# Autodesk Inventor assembly: WheelAssembly3.0
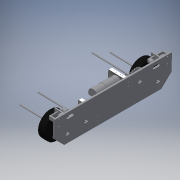
[picture p0: Inventor's stored thumbnail of the model, 180x180]
Saved by Autodesk Inventor 2017 (Build 210142000, 142)
## iProperties
Created: 2017-07-22
Part Number: WheelAssembly3.0
Document SubType Name: Assembly
Designer: User
Author: User
## Documents named in this file (13)
- C:\Robotics\CAD\WheelAssembly3.0.iam
- C:\Robotics\CAD\2016-17_CAD\DriveTrain\DriveTrain3.0.ipt
- C:\Robotics\CAD\COTSParts\Motors\Andymark 2964  NeveRest 40 Motor.ipt
- C:\Robotics\CAD\COTSParts\Tetrix\tetrix-motor-mounts-1.snapshot.1\Tetrex 2pc motor mount.ipt
- C:\Robotics\CAD\COTSParts\Actobotics\615 parts\615398.ipt
- C:\Robotics\CAD\2016-17_CAD\Custom COTS\4inax.ipt
- C:\Robotics\CAD\COTSParts\Actobotics\615 parts\615106.ipt
- C:\Robotics\CAD\COTSParts\Actobotics\545 parts\545556.ipt
- C:\Robotics\CAD\COTSParts\Actobotics\615 parts\615114.ipt
- C:\Robotics\CAD\2016-17_CAD\DriveTrain\Tensioner.iam
- C:\Robotics\CAD\COTSParts\Actobotics\545 parts\545456.ipt
- C:\Robotics\CAD\COTSParts\Wheels\4in Wheel Intergreated Hub 8mm Rev2.ipt
- C:\Robotics\CAD\2016-17_CAD\DriveTrain\MotorFixedPositionMount.ipt
## Components (33 placed, 12 different names)
1. DriveTrain3.0:1 — Flush:3, Flush:4, Mate:2, Flush:5, Mate:3, Flush:6, Angle:1, Insert:7, Insert:8, Angle:2, Insert:9, Insert:10, Insert:16, Insert:17, Mate:6, Flush:9, Flush:10, Mate:12, Mate:13, Flush:12, Flush:13
2. Andymark 2964  NeveRest 40 Motor:1 — Insert:3, Insert:6, Angle:2
3. Andymark 2964  NeveRest 40 Motor:2 — Insert:4, Insert:5, Angle:1
4. Tetrex 2pc motor mount:1 — Insert:3, Flush:3, Mate:3, Flush:6, Mate:17, Insert:32, Insert:33
5. Tetrex 2pc motor mount:2 — Insert:4, Flush:4, Mate:2, Flush:5, Mate:10, Insert:30, Insert:31
6. 615398:1 — Insert:5
7. 615398:2 — Insert:6
8. 615398:3 — Insert:7
9. 615398:4 — Insert:8, Mate:20
10. 4inax:1 — Insert:9, Mate:18
11. 4inax:2 — Insert:10, Mate:8, Mate:16, Mate:19
12. 615106:2 — Insert:26
13. 4inax:3 — Insert:16, Mate:5
14. 4inax:4 — Insert:17, Mate:9, Mate:14, Mate:15
15. 545556:3 — Mate:12, Insert:26, Mate:14, Insert:29
16. 615114:2 — Mate:5, Insert:25
17. 545556:4 — Insert:25
18. Tensioner:1 [sub-assembly] — Mate:6, Flush:9, Flush:10
19. 545556:5 — Insert:23
20. 545456:1 — Insert:23, Insert:24
21. 4in Wheel Intergreated Hub 8mm Rev2:1 — Insert:24
22. DriveTrain3.0:2 — Mate:8, Mate:9, Mate:10
23. Tensioner:2 [sub-assembly] — Mate:13, Flush:12, Flush:13
24. 545556:6 — Insert:27, Insert:29
25. 545456:2 — Insert:27, Insert:28
26. 4in Wheel Intergreated Hub 8mm Rev2:2 — Insert:28
27. DriveTrain3.0:3 — Mate:15, Mate:16, Mate:17
28. MotorFixedPositionMount:1 — Insert:30, Insert:31
29. MotorFixedPositionMount:2 — Insert:32, Insert:33
30. 545556:7 — Insert:34, Mate:18
31. 545556:8 — Insert:35, Mate:19
32. 615114:3 — Insert:34, Mate:20, Flush:16
33. 615106:3 — Insert:35, Flush:16
## Relationships (50: Insert 23, Mate 16, Flush 9, Angle 2)
- Insert:3: Andymark 2964  NeveRest 40 Motor:1 ↔ Tetrex 2pc motor mount:1
- Insert:4: Andymark 2964  NeveRest 40 Motor:2 ↔ Tetrex 2pc motor mount:2
- Flush:3 (159.5374 mm): DriveTrain3.0:1 ↔ Tetrex 2pc motor mount:1
- Flush:4 (159.5374 mm): DriveTrain3.0:1 ↔ Tetrex 2pc motor mount:2
- Insert:5: Andymark 2964  NeveRest 40 Motor:2 ↔ 615398:1
- Mate:2: DriveTrain3.0:1 ↔ Tetrex 2pc motor mount:2
- Flush:5 (7.3152 mm): DriveTrain3.0:1 ↔ Tetrex 2pc motor mount:2
- Mate:3: DriveTrain3.0:1 ↔ Tetrex 2pc motor mount:1
- Flush:6 (-20.3454 mm): DriveTrain3.0:1 ↔ Tetrex 2pc motor mount:1
- Angle:1 (0 deg): DriveTrain3.0:1 ↔ Andymark 2964  NeveRest 40 Motor:2
- Insert:6: Andymark 2964  NeveRest 40 Motor:1 ↔ 615398:2
- Insert:7 (25.4508 mm): DriveTrain3.0:1 ↔ 615398:3
- Insert:8 (25.4508 mm): DriveTrain3.0:1 ↔ 615398:4
- Angle:2 (180 deg): DriveTrain3.0:1 ↔ Andymark 2964  NeveRest 40 Motor:1
- Insert:9 (-6.35 mm): DriveTrain3.0:1 ↔ 4inax:1
- Insert:10 (-6.35 mm): DriveTrain3.0:1 ↔ 4inax:2
- Insert:16 (-6.35 mm): DriveTrain3.0:1 ↔ 4inax:3
- Insert:17 (-6.35 mm): DriveTrain3.0:1 ↔ 4inax:4
- Mate:5: 4inax:3 ↔ 615114:2
- Mate:6: DriveTrain3.0:1 ↔ Tensioner:1
- Flush:9 (34.925 mm): DriveTrain3.0:1 ↔ Tensioner:1
- Flush:10: DriveTrain3.0:1 ↔ Tensioner:1
- Insert:23: 545556:5 ↔ 545456:1
- Insert:24: 545456:1 ↔ 4in Wheel Intergreated Hub 8mm Rev2:1
- Mate:8: 4inax:2 ↔ DriveTrain3.0:2
- Mate:9: 4inax:4 ↔ DriveTrain3.0:2
- Mate:10: Tetrex 2pc motor mount:2 ↔ DriveTrain3.0:2
- Mate:12 (3.175 mm): DriveTrain3.0:1 ↔ 545556:3
- Mate:13: DriveTrain3.0:1 ↔ Tensioner:2
- Flush:12 (34.925 mm): DriveTrain3.0:1 ↔ Tensioner:2
- Flush:13: DriveTrain3.0:1 ↔ Tensioner:2
- Insert:25: 615114:2 ↔ 545556:4
- Insert:26: 615106:2 ↔ 545556:3
- Mate:14: 4inax:4 ↔ 545556:3
- Insert:27: 545556:6 ↔ 545456:2
- Insert:28: 545456:2 ↔ 4in Wheel Intergreated Hub 8mm Rev2:2
- Insert:29 (9.144 mm): 545556:3 ↔ 545556:6
- Mate:15: 4inax:4 ↔ DriveTrain3.0:3
- Mate:16: 4inax:2 ↔ DriveTrain3.0:3
- Mate:17: Tetrex 2pc motor mount:1 ↔ DriveTrain3.0:3
- Insert:30: Tetrex 2pc motor mount:2 ↔ MotorFixedPositionMount:1
- Insert:31: Tetrex 2pc motor mount:2 ↔ MotorFixedPositionMount:1
- Insert:32: Tetrex 2pc motor mount:1 ↔ MotorFixedPositionMount:2
- Insert:33: Tetrex 2pc motor mount:1 ↔ MotorFixedPositionMount:2
- Insert:34: 545556:7 ↔ 615114:3
- Insert:35: 545556:8 ↔ 615106:3
- Mate:18: 4inax:1 ↔ 545556:7
- Mate:19: 4inax:2 ↔ 545556:8
- Mate:20: 615398:4 ↔ 615114:3
- Flush:16: 615114:3 ↔ 615106:3
